# Autodesk Inventor assembly: 536270 ADN-32-15-A-P-A---(asm_0)
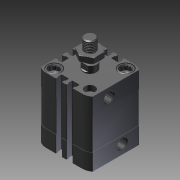
[picture p0: Inventor's stored thumbnail of the model, 180x180]
Saved by Autodesk Inventor 2011 SP1 (Build 150282100, 282)
## iProperties
Created: 2018-05-26
Part Number: 536270 ADN-32-15-A-P-A---(asm_0)
Catalog Web Link: www.cadenas.de
Description: ADN-Compact cylinder
Vendor: FESTO
Document SubType Name: Assembly
Designer: psAdmin
Manufacturer: FESTO
Mass: 310 g
Category: PARTsolutions
Company: FESTO
Title: 536270 ADN-32-15-A-P-A
Author: Cadenas PARTsolutions
Comments: Compact cylinder
PSOL_IDENT_0: {$CADENAS_DATA\23d-libs\festo\parts\a\adn\adn_std_tab.prj},213 {VTYP=3D},{STYP=ASSTAB},{NB=536270 AD
PSOL_IDENT_1: N-32-15-A-P-A---(asm_0)},{LINA=536270 ADN-32-15-A-P-A},{NN=ADN},{DATE=17.05.2018 10:40:18},{GEOMDATE=
PSOL_IDENT_2: 24.04.2017 11:47:47},{VERSION=},{LINEID=440},{LINESUBID=-1},{WBVAR=HUBST}  {NB=536270 ADN-32-15-A-P-
PSOL_IDENT_3: A---(asm_0)},{LINA=536270 ADN-32-15-A-P-A},{KT=DUMMY},{TNR=536270},{TYP=ADN-32-15-A-P-A},{KDM=32},{H
PSOL_IDENT_4: UB=15},{HUBST=0},{DF=P},{TH=A},{Q=0},{S2=0},{K2=0},{K5=0},{K8=0},{ZZ=0},{A=19.000},{AF=16.000},{BG=2
PSOL_IDENT_5: 7.000},{D1=9.000},{D5=9.000},{E=47.000},{EE=G1/8},{EEN=9.728},{EEK=8.566},{G=15.000},{KF=M8},{KFN=8.
PSOL_IDENT_6: 000},{KFK=6.647},{KFNW=8},{KFKW=6.647},{KK=M10x1.25},{KKN=10.000},{KKK=8.160},{KKNW=10},{KKKW=8.16},
PSOL_IDENT_7: {L3=5.000},{L12=4.700},{MM=12.000},{PL=8.200},{RR=5.100},{RT=M6},{RTN=6.000},{RTK=4.917},{SW=10.000}
PSOL_IDENT_8: ,{T1=2.100},{T4=3.300},{TG=32.500},{WH=6.000},{ZA=44.000},{ZB=50.000},{J3=6.000},{SWQ=10.000},{RA=9.
PSOL_IDENT_9: 700},{RU=35.200},{RT1=3.400},{RB1=5.400},{RB2=6.800},{R1=12.400},{R2=1.000},{FORM=2},{MASSBKS=0.060}
PSOL_IDENT_10: ,{MASSHKS=0.009},{MASSBZR=0.265},{MASSHZR=0.030},{CNSMASSEXACT=0.31},{PPATH=assemblies/adn_asmtpl.pr
PSOL_IDENT_11: j}
NN: ADN
NT: Compact cylinder
NB: 536270 ADN-32-15-A-P-A---(asm_0)
NBSYN: $TNR. $TYP.---(asm_$HUBST.)
LINA: 536270 ADN-32-15-A-P-A
OFFICIAL_STANDARD_NUMBERS: ISO 21287
TNR: 536270
TYP: ADN-32-15-A-P-A
KDM: 32
HUB: 15
HUBST: 0
DF: P
TH: A
A: 19.000
AF: 16.000
BG: 27.000
D1: 9.000
D5: 9.000
E: 47.000
EE: G1/8
G: 15.000
KF: M8
KK: M10x1.25
L3: 5.000
L12: 4.700
MM: 12.000
PL: 8.200
RR: 5.100
RT: M6
SW: 10.000
T1: 2.100
T4: 3.300
TG: 32.500
WH: 6.000
ZA: 44.000
ZB: 50.000
J3: 6.000
RA: 9.700
RU: 35.200
R1: 12.400
R2: 1.000
CNSMASSEXACT: 0.310
SUPPLIER: FESTO
ARTICLENO: 536270 ADN-32-15-A-P-A---(asm_0)
BOMINFO: 536270 ADN-32-15-A-P-A
CREATOR: CADENAS GmbH
## Documents named in this file (4)
- p:\temp\worker_2\836_452\cad_40_02018052614550788843352192d056f_000000_00_00_000001\536270 ADN-32-15-A-P-A---(asm_0).iam
- p:\temp\worker_2\836_452\cad_40_02018052614550788843352192d056f_000000_00_00_000001\536267 ADN-15-P---(Z).ipt
- p:\temp\worker_2\836_452\cad_40_02018052614550788843352192d056f_000000_00_00_000001\536267 ADN-15-P-A_(KS).ipt
- p:\temp\worker_2\836_452\cad_40_02018052614550788843352192d056f_000000_00_00_000001\DIN-439-B - M10x1_25(F).ipt
## Components (3 placed, 3 different names)
1. 536267 ADN-15-P---(Z):1 — CYLINDER_Z@1 <-> PISTON_Z@2, CYLINDER_YZ@1 <-> PISTON_YZ@2
2. 536267 ADN-15-P-A_(KS):1 — CYLINDER_Z@1 <-> PISTON_Z@2, CYLINDER_YZ@1 <-> PISTON_YZ@2, NUT1_XY@2 <-> 2CYL_XY@3, NUT1_Z@2 <-> 2CYL_Z@3, NUT1_YZ@2 <-> 2CYL_YZ@3
3. DIN-439-B - M10x1_25(F):1 — NUT1_XY@2 <-> 2CYL_XY@3, NUT1_Z@2 <-> 2CYL_Z@3, NUT1_YZ@2 <-> 2CYL_YZ@3
## Relationships (5: Mate 3, Angle 2)
- CYLINDER_Z@1 <-> PISTON_Z@2 [Mate]: 536267 ADN-15-P---(Z):1 ↔ 536267 ADN-15-P-A_(KS):1
- CYLINDER_YZ@1 <-> PISTON_YZ@2 [Angle] (0 deg): 536267 ADN-15-P---(Z):1 ↔ 536267 ADN-15-P-A_(KS):1
- NUT1_XY@2 <-> 2CYL_XY@3 [Mate]: 536267 ADN-15-P-A_(KS):1 ↔ DIN-439-B - M10x1_25(F):1
- NUT1_Z@2 <-> 2CYL_Z@3 [Mate]: 536267 ADN-15-P-A_(KS):1 ↔ DIN-439-B - M10x1_25(F):1
- NUT1_YZ@2 <-> 2CYL_YZ@3 [Angle] (0 deg): 536267 ADN-15-P-A_(KS):1 ↔ DIN-439-B - M10x1_25(F):1
